# Autodesk Inventor assembly: wheel sub assemblly omni wheel
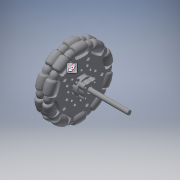
[picture p0: Inventor's stored thumbnail of the model, 180x180]
Saved by Autodesk Inventor 2017 (Build 210142000, 142)
## iProperties
Created: 2017-08-02
Part Number: wheel sub assemblly omni wheel
Document SubType Name: Assembly
Designer: User
Author: User
## Documents named in this file (6)
- C:\Robotics\CAD\2016-17_CAD\DriveTrain\wheel sub assemblly omni wheels.iam
- C:\Robotics\CAD\COTSParts\Actobotics\634 parts\634080.ipt
- C:\Robotics\CAD\COTSParts\Actobotics\545 parts\545556.ipt
- C:\Robotics\CAD\COTSParts\Actobotics\545 parts\545456.ipt
- C:\Robotics\CAD\COTSParts\Actobotics\615 parts\615106.ipt
- C:\Robotics\CAD\COTSParts\595671 Part.ipt
## Components (7 placed, 5 different names)
1. 634080:1 — Mate:9, Mate:10
2. 545556:1 — Mate:13, Mate:14
3. 545556:2
4. 545456:1 — Mate:12
5. 615106:1 — Mate:13
6. 595671 Part:1 — Mate:9, Mate:11, Mate:14
7. 595671 Part:3 — Mate:10, Mate:11, Mate:12
## Relationships (11: Mate 11)
- [Mate]: 545556:1 ↔ 615106:1
- [Mate]: 634080:1 ↔ 545456:1
- [Mate]: 634080:1 ↔ 545556:2
- [Mate]: 545556:2 ↔ 545456:1
- [Mate]: 634080:1 ↔ 545556:1
- Mate:9: 634080:1 ↔ 595671 Part:1
- Mate:10: 634080:1 ↔ 595671 Part:3
- Mate:11: 595671 Part:1 ↔ 595671 Part:3
- Mate:12: 545456:1 ↔ 595671 Part:3
- Mate:13: 545556:1 ↔ 615106:1
- Mate:14: 545556:1 ↔ 595671 Part:1
